# Autodesk Inventor assembly: Mk.2
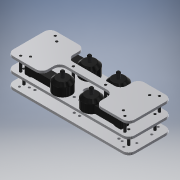
[picture p0: Inventor's stored thumbnail of the model, 180x180]
Saved by Autodesk Inventor 2019 (Build 230136000, 136)
## iProperties
Created: 2019-10-24
Part Number: Mk.2
Document SubType Name: Assembly
Designer: robgr
Author: robgr
## Documents named in this file (7)
- C:\Users\robgr\Desktop\Drone Shit\Models\Mk.2.iam
- C:\Users\robgr\Desktop\Drone Shit\Models\Base Plate New.ipt
- C:\Users\robgr\Desktop\Drone Shit\Models\support rods.ipt
- C:\Users\robgr\Desktop\Drone Shit\Models\top plate.ipt
- C:\Users\robgr\Desktop\Drone Shit\Models\Motor.ipt
- C:\Users\robgr\Desktop\Drone Shit\Models\frontside arm.ipt
- C:\Users\robgr\Desktop\Drone Shit\Models\motorstop.ipt
## Components (25 placed, 6 different names)
1. Base Plate New:2 — Mate:1, Mate:2, Mate:3, Mate:4, Flush:1, Flush:2, Flush:3, Flush:4, Mate:65, Mate:66, Flush:13, Flush:14, Flush:15, Flush:16, Flush:21, Mate:73, Mate:74
2. support rods:1 — Mate:1, Flush:4, Flush:6, Mate:22
3. support rods:2 — Mate:2, Flush:3, Mate:55
4. support rods:3 — Mate:3, Flush:1, Mate:9, Mate:12
5. support rods:4 — Mate:4, Flush:2, Mate:10, Mate:11
6. top plate:1 — Flush:6, Mate:9, Mate:10, Angle:1, Angle:4, Angle:5, Mate:59, Flush:7, Flush:9, Mate:60, Mate:61, Mate:62, Flush:11, Flush:12, Mate:69, Mate:70, Mate:71, Mate:72, Angle:6, Mate:75, Flush:22, Mate:76, Flush:23
7. Motor:1 — Mate:26, Mate:27, Mate:28
8. Motor:2 — Mate:19, Mate:20, Mate:21
9. Motor:3 — Mate:29, Mate:30, Mate:31
10. frontside arm:1 — Mate:12, Mate:19, Mate:20, Mate:21, Angle:4, Mate:72
11. frontside arm:2 — Mate:11, Mate:29, Mate:30, Mate:31, Mate:69, Angle:6
12. frontside arm:4 — Mate:22, Mate:26, Mate:27, Mate:28, Angle:1, Mate:71
13. frontside arm:5 — Mate:55, Mate:56, Mate:57, Mate:58, Angle:5, Mate:70
14. Motor:4 — Mate:56, Mate:57, Mate:58
15. motorstop:1 — Mate:61, Flush:12
16. motorstop:2 — Mate:62, Flush:11
17. motorstop:3 — Mate:59, Flush:7
18. motorstop:4 — Flush:9, Mate:60
19. Base Plate New:3 — Mate:67, Mate:68, Flush:17, Flush:18, Flush:19, Flush:20
20. support rods:5 — Mate:66, Flush:14, Flush:20
21. support rods:6 — Flush:16, Mate:68, Flush:17, Flush:21, Mate:73
22. support rods:7 — Mate:65, Flush:13, Flush:19
23. support rods:8 — Flush:15, Mate:67, Flush:18, Mate:74
24. support rods:9 — Mate:75, Flush:22
25. support rods:10 — Mate:76, Flush:23
## Relationships (62: Mate 38, Flush 20, Angle 4)
- Mate:1: Base Plate New:2 ↔ support rods:1
- Mate:2: Base Plate New:2 ↔ support rods:2
- Mate:3: Base Plate New:2 ↔ support rods:3
- Mate:4: Base Plate New:2 ↔ support rods:4
- Flush:1: Base Plate New:2 ↔ support rods:3
- Flush:2: Base Plate New:2 ↔ support rods:4
- Flush:3: Base Plate New:2 ↔ support rods:2
- Flush:4: Base Plate New:2 ↔ support rods:1
- Flush:6: support rods:1 ↔ top plate:1
- Mate:9: support rods:3 ↔ top plate:1
- Mate:10: support rods:4 ↔ top plate:1
- Mate:11: support rods:4 ↔ frontside arm:2
- Mate:12: support rods:3 ↔ frontside arm:1
- Mate:19: Motor:2 ↔ frontside arm:1
- Mate:20: Motor:2 ↔ frontside arm:1
- Mate:21: Motor:2 ↔ frontside arm:1
- Mate:22: support rods:1 ↔ frontside arm:4
- Mate:26: Motor:1 ↔ frontside arm:4
- Mate:27: Motor:1 ↔ frontside arm:4
- Mate:28: Motor:1 ↔ frontside arm:4
- Mate:29: Motor:3 ↔ frontside arm:2
- Mate:30: Motor:3 ↔ frontside arm:2
- Mate:31: Motor:3 ↔ frontside arm:2
- Angle:1 (0 deg): top plate:1 ↔ frontside arm:4
- Angle:4 (0 deg): top plate:1 ↔ frontside arm:1
- Mate:55: support rods:2 ↔ frontside arm:5
- Mate:56: frontside arm:5 ↔ Motor:4
- Mate:57: frontside arm:5 ↔ Motor:4
- Mate:58: frontside arm:5 ↔ Motor:4
- Angle:5 (0 deg): top plate:1 ↔ frontside arm:5
- Mate:59: top plate:1 ↔ motorstop:3
- Flush:7: top plate:1 ↔ motorstop:3
- Flush:9: top plate:1 ↔ motorstop:4
- Mate:60: top plate:1 ↔ motorstop:4
- Mate:61: top plate:1 ↔ motorstop:1
- Mate:62: top plate:1 ↔ motorstop:2
- Flush:11: top plate:1 ↔ motorstop:2
- Flush:12: top plate:1 ↔ motorstop:1
- Mate:65: Base Plate New:2 ↔ support rods:7
- Mate:66: Base Plate New:2 ↔ support rods:5
- Flush:13: Base Plate New:2 ↔ support rods:7
- Flush:14: Base Plate New:2 ↔ support rods:5
- Flush:15: Base Plate New:2 ↔ support rods:8
- Flush:16: Base Plate New:2 ↔ support rods:6
- Mate:67: Base Plate New:3 ↔ support rods:8
- Mate:68: Base Plate New:3 ↔ support rods:6
- Flush:17: Base Plate New:3 ↔ support rods:6
- Flush:18: Base Plate New:3 ↔ support rods:8
- Flush:19: Base Plate New:3 ↔ support rods:7
- Flush:20: Base Plate New:3 ↔ support rods:5
- Mate:69: top plate:1 ↔ frontside arm:2
- Mate:70: top plate:1 ↔ frontside arm:5
- Mate:71: top plate:1 ↔ frontside arm:4
- Mate:72: top plate:1 ↔ frontside arm:1
- Angle:6 (0 deg): top plate:1 ↔ frontside arm:2
- Flush:21: Base Plate New:2 ↔ support rods:6
- Mate:73: Base Plate New:2 ↔ support rods:6
- Mate:74: Base Plate New:2 ↔ support rods:8
- Mate:75: top plate:1 ↔ support rods:9
- Flush:22: top plate:1 ↔ support rods:9
- Mate:76: top plate:1 ↔ support rods:10
- Flush:23: top plate:1 ↔ support rods:10
